# Autodesk Inventor assembly: A-00-0
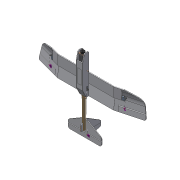
[picture p0: Inventor's stored thumbnail of the model, 180x180]
Saved by Autodesk Inventor 2019 (Build 230136000, 136)
## iProperties
Created: 2022-04-09
Part Number: A-00-0
Document SubType Name: Assembly
Designer: solyo
Mass: 180.687 g
Surface Area: 4241.02 cm^2
Volume: 1031.39 cm^3
Density: 0.175188 g/cm^3
Author: solyo
## Documents named in this file (23)
- D:\Modelling\RC\RC Trainer V1\Design\Assembly\A-03-0-ONE_LEVEL\A-04-0.iam
- D:\Modelling\RC\RC Trainer V1\Design\Parts\PW-00-0-TAILBOOM\PW-00-0-0.ipt
- D:\Modelling\RC\RC Trainer V1\Design\Parts\PW-01-0-FIREWALL\PW-01-0-0.ipt
- D:\Modelling\RC\RC Trainer V1\Design\Parts\PW-02-0-PIN\PW-02-0-0\WING_FRONT_TIE.ipt
- D:\Modelling\RC\RC Trainer V1\Design\Parts\PW-02-0-PIN\PW-02-0-0\WING_REAR_TIE.ipt
- D:\Modelling\RC\RC Trainer V1\Design\Parts\PF-01-0-FUSELAGE\PF-01-0-1.ipt
- D:\Modelling\RC\RC Trainer V1\Design\Parts\C-01-0-EMAX_MT1806_2280KV\C-01-0.ipt
- D:\Modelling\RC\RC Trainer V1\Design\Parts\PF-02-0-HORIZONTAL_STABILIZER\PF-02-0-0.ipt
- D:\Modelling\RC\RC Trainer V1\Design\Parts\PF-03-0-VERTICAL_STABILIZER\PF-03-0-0.ipt
- D:\Modelling\RC\RC Trainer V1\Design\Parts\PW-02-0-PIN\PW-02-0-0\SLIDE.ipt
- D:\Modelling\RC\RC Trainer V1\Design\Parts\C-00-0-BATTERY_600MAH\C-00-0.ipt
- D:\Modelling\RC\RC Trainer V1\Design\Parts\C-03-0-SERVO_3G\C-03-0\CW.ipt
- D:\Modelling\RC\RC Trainer V1\Design\Parts\PP-00-0-CONTROL_HORN\PP-00-0-0.ipt
- D:\Modelling\RC\RC Trainer V1\Design\Parts\C-02-0-EMAX_12AESC\C-02-0.ipt
- D:\Modelling\RC\RC Trainer V1\Design\Parts\PF-00-0-WING\PF-00-0-1.ipt
- D:\Modelling\RC\RC Trainer V1\Design\Parts\C-03-0-SERVO_3G\C-03-0\CCW.ipt
- D:\Modelling\RC\Microplane\Design\Parts\C-03-0-SERVO_3G\C-03-0.ipt
- D:\Modelling\RC\RC Trainer V1\Design\Parts\PM-00-0-PUSHROD\PM-00-0-0\AILERON.ipt
- D:\Modelling\RC\Microplane\Design\Parts\PM-00-0-PUSHROD\PM-00-0-0.ipt
- D:\Modelling\RC\RC Trainer V1\Design\Parts\PM-00-0-PUSHROD\PM-00-0-0\TAIL.ipt
- D:\Modelling\RC\RC Trainer V1\Design\Parts\PW-02-0-PIN\PW-02-0-0.ipt
- D:\Modelling\RC\RC Trainer V1\Design\Parts\C-03-0-SERVO_3G\C-03-0.ipt
- D:\Modelling\RC\RC Trainer V1\Design\Parts\C-04-0-SERVO_LINKAGE_STOPPER\C-04-0.ipt
## Components (28 placed, 18 different names)
1. PW-00-0-0:1 — Flush:1, Flush:2, Flush:3, Mate:1, Flush:5, Mate:6, Mate:13, Mate:14, Mate:15, Mate:32, Mate:44, Mate:45, Insert:15, Insert:16
2. PW-01-0-0:1 — Flush:4, Mate:1, Flush:5, Mate:8, Insert:1, Mate:9, Mate:20, Mate:60
3. WING_FRONT_TIE:1 — Insert:15, Mate:59
4. WING_REAR_TIE:2 — Insert:16
5. PF-01-0-1:1 — Mate:6, Mate:8, Mate:19, Flush:15, Flush:16, Mate:43, Mate:46, Mate:47, Mate:48, Mate:50, Mate:59
6. C-01-0:1 — Insert:1, Mate:9
7. PF-02-0-0:1 — Mate:10, Mate:11, Mate:12, Mate:14, Mate:25, Mate:26, Mate:49
8. PF-03-0-0:1 — Mate:10, Mate:11, Mate:12, Mate:13, Mate:15, Mate:17, Flush:6, Mate:28, Mate:29, Mate:61
9. SLIDE:4 — Mate:17, Flush:6, Mate:61
10. C-00-0:1 — Mate:18, Mate:19, Mate:20
11. TAIL:5 — Mate:56, Mate:57, Mate:58
12. TAIL:6 — Mate:62, Mate:63, Mate:64, Mate:65, Mate:66
13. PP-00-0-0:1 — Mate:25, Mate:26, Insert:14
14. PP-00-0-0:2 — Mate:28, Mate:29, Mate:49, Insert:13
15. C-02-0:2 — Mate:31, Mate:32, Mate:60
16. PF-00-0-1:1 — Mate:33, Mate:35, Flush:15, Flush:16, Mate:43, Flush:17, Mate:52, Flush:18, Mate:53
17. CCW:7 — Mate:33, Flush:17, Mate:52, Insert:9
18. CW:4 — Mate:35, Mate:42, Flush:18, Mate:53, Insert:10
19. PP-00-0-0:3 — Insert:11
20. PP-00-0-0:4 — Insert:8
21. AILERON:3 — Insert:9, Mate:54
22. AILERON:4 — Mate:42, Insert:10, Mate:55
23. CW:5 — Mate:44, Mate:47, Mate:50, Mate:62, Mate:63, Mate:65
24. CW:6 — Mate:45, Mate:48, Mate:46, Mate:57, Mate:58
25. C-04-0:1 — Insert:8, Mate:54
26. C-04-0:2 — Insert:11, Mate:55
27. C-04-0:3 — Insert:13, Mate:64, Mate:66
28. C-04-0:5 — Insert:14, Mate:56
## Relationships (70: Mate 51, Flush 10, Insert 9)
- Flush:1: PW-00-0-0:1
- Flush:2: PW-00-0-0:1
- Flush:3: PW-00-0-0:1
- Flush:4: PW-01-0-0:1
- Mate:1: PW-00-0-0:1 ↔ PW-01-0-0:1
- Flush:5: PW-00-0-0:1 ↔ PW-01-0-0:1
- Mate:6: PW-00-0-0:1 ↔ PF-01-0-1:1
- Mate:8: PW-01-0-0:1 ↔ PF-01-0-1:1
- Insert:1: PW-01-0-0:1 ↔ C-01-0:1
- Mate:9: PW-01-0-0:1 ↔ C-01-0:1
- Mate:10: PF-02-0-0:1 ↔ PF-03-0-0:1
- Mate:11: PF-02-0-0:1 ↔ PF-03-0-0:1
- Mate:12: PF-02-0-0:1 ↔ PF-03-0-0:1
- Mate:13: PW-00-0-0:1 ↔ PF-03-0-0:1
- Mate:14: PW-00-0-0:1 ↔ PF-02-0-0:1
- Mate:15: PW-00-0-0:1 ↔ PF-03-0-0:1
- Mate:17 (-2.5 mm): PF-03-0-0:1 ↔ SLIDE:4
- Flush:6: PF-03-0-0:1 ↔ SLIDE:4
- Mate:18: C-00-0:1
- Mate:19: PF-01-0-1:1 ↔ C-00-0:1
- Mate:20: PW-01-0-0:1 ↔ C-00-0:1
- Mate:25: PF-02-0-0:1 ↔ PP-00-0-0:1
- Mate:26: PF-02-0-0:1 ↔ PP-00-0-0:1
- Mate:28: PF-03-0-0:1 ↔ PP-00-0-0:2
- Mate:29: PF-03-0-0:1 ↔ PP-00-0-0:2
- Mate:31: C-02-0:2
- Mate:32: PW-00-0-0:1 ↔ C-02-0:2
- Mate:33: PF-00-0-1:1 ↔ CCW:7
- Mate:35: PF-00-0-1:1 ↔ CW:4
- [Mate]: PF-00-0-1:1 ↔ PP-00-0-0:3
- [Mate]: PF-00-0-1:1 ↔ PP-00-0-0:3
- [Mate]: PF-00-0-1:1 ↔ PP-00-0-0:4
- [Mate]: PF-00-0-1:1 ↔ PP-00-0-0:4
- [Mate]: CCW:7 ↔ AILERON:3
- Mate:42: CW:4 ↔ AILERON:4
- Flush:15: PF-01-0-1:1 ↔ PF-00-0-1:1
- Flush:16: PF-01-0-1:1 ↔ PF-00-0-1:1
- Mate:43: PF-01-0-1:1 ↔ PF-00-0-1:1
- Mate:44: PW-00-0-0:1 ↔ CW:5
- Mate:47: PF-01-0-1:1 ↔ CW:5
- Mate:45: PW-00-0-0:1 ↔ CW:6
- Mate:48: PF-01-0-1:1 ↔ CW:6
- Mate:46: PF-01-0-1:1 ↔ CW:6
- Mate:49 (10 mm): PF-02-0-0:1 ↔ PP-00-0-0:2
- Mate:50: PF-01-0-1:1 ↔ CW:5
- Flush:17: PF-00-0-1:1 ↔ CCW:7
- Mate:52: PF-00-0-1:1 ↔ CCW:7
- Flush:18: PF-00-0-1:1 ↔ CW:4
- Mate:53: PF-00-0-1:1 ↔ CW:4
- Insert:8: PP-00-0-0:4 ↔ C-04-0:1
- Insert:9 (1 mm): CCW:7 ↔ AILERON:3
- Mate:54: AILERON:3 ↔ C-04-0:1
- Insert:10 (1 mm): CW:4 ↔ AILERON:4
- Insert:11: PP-00-0-0:3 ↔ C-04-0:2
- Mate:55: AILERON:4 ↔ C-04-0:2
- Insert:13: PP-00-0-0:2 ↔ C-04-0:3
- Insert:14: PP-00-0-0:1 ↔ C-04-0:5
- Mate:56: TAIL:5 ↔ C-04-0:5
- Mate:57: TAIL:5 ↔ CW:6
- Mate:58 (1 mm): TAIL:5 ↔ CW:6
- Insert:15 (-26 mm): PW-00-0-0:1 ↔ WING_FRONT_TIE:1
- Mate:59: WING_FRONT_TIE:1 ↔ PF-01-0-1:1
- Insert:16 (-20 mm): PW-00-0-0:1 ↔ WING_REAR_TIE:2
- Mate:60: PW-01-0-0:1 ↔ C-02-0:2
- Mate:61: PF-03-0-0:1 ↔ SLIDE:4
- Mate:62: TAIL:6 ↔ CW:5
- Mate:63 (1 mm): TAIL:6 ↔ CW:5
- Mate:64: TAIL:6 ↔ C-04-0:3
- Mate:65: TAIL:6 ↔ CW:5
- Mate:66: TAIL:6 ↔ C-04-0:3
## Named parameters: d55_d6 = 0 mm, d58_d9 = 0 mm, d60_d11 = 0 mm, d61_d12 = 0 mm, d63_d14 = 0 mm, d66_d17 = 0 mm, d67_d18 = 0 mm
